# Autodesk Inventor assembly: Сборка1
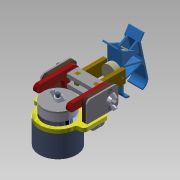
[picture p0: Inventor's stored thumbnail of the model, 180x180]
Saved by Autodesk Inventor 2018 (Build 220112000, 112)
## iProperties
Created: 2020-02-22
Part Number: Сборка1
Material: Типовые
Document SubType Name: Assembly
Designer: Leancher
Mass: 129.322 g
Surface Area: 473.979 cm^2
Volume: 129.322 cm^3
Density: 1 g/cm^3
Author: Leancher
## Documents named in this file (19)
- C:\Users\Leancher\GoogleDrive\My_project\Механика\Фотоштатив\Сборка1.iam
- C:\Users\Leancher\GoogleDrive\My_project\Механика\Фотоштатив\Гор. шарнир.ipt
- C:\Users\Leancher\GoogleDrive\My_project\Механика\Фотоштатив\Верт. держатели.ipt
- C:\Users\Leancher\GoogleDrive\My_project\Механика\Фотоштатив\В.шарн. - втулка.ipt
- C:\Users\Leancher\GoogleDrive\My_project\Механика\Фотоштатив\В. шарн. - держатель соединителя.ipt
- C:\Users\Leancher\GoogleDrive\My_project\Механика\Фотоштатив\В. шарн. - соединитель.ipt
- C:\Users\Leancher\GoogleDrive\My_project\Механика\Фотоштатив\В. шарн. - держатель смартфона.ipt
- C:\Users\Leancher\GoogleDrive\My_project\Механика\Фотоштатив\Чертежи\Гор. шарн. - проставка 1.ipt
- C:\Users\Leancher\GoogleDrive\My_project\Механика\Фотоштатив\Чертежи\Гор. шарн. - прижим.ipt
- C:\Users\Leancher\GoogleDrive\My_project\Механика\Фотоштатив\Чертежи\Верх. часть штатива.ipt
- C:\Users\Leancher\GoogleDrive\My_project\Механика\Фотоштатив\Винт М3х10.ipt
- C:\Users\Leancher\GoogleDrive\My_project\Механика\Фотоштатив\Болт М5х16.ipt
- C:\Users\Leancher\GoogleDrive\My_project\Механика\Фотоштатив\Винт М3х6 пот.ipt
- C:\Users\Leancher\GoogleDrive\My_project\Механика\Фотоштатив\Верт держатели-2 левый.ipt
- C:\Users\Leancher\GoogleDrive\My_project\Механика\Фотоштатив\Верт держатели-2 правый.ipt
- C:\Users\Leancher\GoogleDrive\My_project\Механика\Фотоштатив\Гайка М3.ipt
- C:\Users\Leancher\GoogleDrive\My_project\Механика\Фотоштатив\Гайка-барашек М5.ipt
- C:\Users\Leancher\GoogleDrive\My_project\Механика\Фотоштатив\Прищепка смартфона.ipt
- C:\Users\Leancher\GoogleDrive\My_project\Механика\Фотоштатив\Винт М3х30.ipt
## Components (31 placed, 18 different names)
1. Гор. шарнир:1 — Заподлицо:1, Заподлицо:3
2. Верт. держатели:1 — Вставка:1, Совмещение:27
3. Верт. держатели:2 — Вставка:2, Совмещение:28
4. В.шарн. - втулка:1 — Вставка:2, Совмещение:6, Совмещение:7, Заподлицо:6, Совмещение:21
5. В.шарн. - втулка:2 — Вставка:1, Совмещение:4, Совмещение:5, Совмещение:19, Совмещение:20, Совмещение:22
6. В. шарн. - держатель соединителя:1 — Совмещение:4, Совмещение:5, Совмещение:11
7. В. шарн. - держатель соединителя:2 — Совмещение:6, Совмещение:7, Совмещение:8, Совмещение:9, Совмещение:10
8. В. шарн. - соединитель:1 — Совмещение:8, Совмещение:9, Совмещение:13, Совмещение:14, Совмещение:15, Совмещение:16
9. В. шарн. - соединитель:2 — Совмещение:10, Совмещение:11
10. В. шарн. - держатель смартфона:1 — Совмещение:13, Совмещение:14, Совмещение:32
11. В. шарн. - держатель смартфона:2 — Совмещение:15, Совмещение:16, Совмещение:33
12. Гор. шарн. - проставка 1:1 — Заподлицо:1, Заподлицо:2
13. Гор. шарн. - прижим:1 — Заподлицо:2, Совмещение:31
14. Верх. часть штатива:1 — Заподлицо:3
15. Винт М3х10:1 — Совмещение:25
16. Болт М5х16:1 — Заподлицо:6
17. Болт М5х16:2 — Совмещение:19, Совмещение:20
18. Винт М3х6 пот:1
19. Винт М3х6 пот:2
20. Верт держатели-2 левый:1 — Совмещение:21, Совмещение:23, Заподлицо:7, Совмещение:24, Заподлицо:8, Совмещение:26, Совмещение:30
21. Верт держатели-2 правый:1 — Совмещение:22, Совмещение:25, Совмещение:29
22. Винт М3х6 пот:3 — Совмещение:23, Заподлицо:7
23. Винт М3х6 пот:4 — Совмещение:24, Заподлицо:8
24. Винт М3х10:2 — Совмещение:26
25. Гайка М3:1 — Совмещение:27
26. Гайка М3:2 — Совмещение:28
27. Гайка-барашек М5:1 — Совмещение:31
28. Гайка-барашек М5:2 — Совмещение:29
29. Гайка-барашек М5:3 — Совмещение:30
30. Прищепка смартфона:1 — Совмещение:32
31. Винт М3х30:1 — Совмещение:33
## Relationships (35: Mate 27, Flush 6, Insert 2)
- Вставка:1 [Insert]: Верт. держатели:1 ↔ В.шарн. - втулка:2
- Вставка:2 [Insert]: Верт. держатели:2 ↔ В.шарн. - втулка:1
- Совмещение:4 [Mate]: В.шарн. - втулка:2 ↔ В. шарн. - держатель соединителя:1
- Совмещение:5 [Mate]: В.шарн. - втулка:2 ↔ В. шарн. - держатель соединителя:1
- Совмещение:6 [Mate]: В.шарн. - втулка:1 ↔ В. шарн. - держатель соединителя:2
- Совмещение:7 [Mate]: В.шарн. - втулка:1 ↔ В. шарн. - держатель соединителя:2
- Совмещение:8 [Mate]: В. шарн. - держатель соединителя:2 ↔ В. шарн. - соединитель:1
- Совмещение:9 [Mate]: В. шарн. - держатель соединителя:2 ↔ В. шарн. - соединитель:1
- Совмещение:10 [Mate]: В. шарн. - держатель соединителя:2 ↔ В. шарн. - соединитель:2
- Совмещение:11 [Mate]: В. шарн. - держатель соединителя:1 ↔ В. шарн. - соединитель:2
- Совмещение:13 [Mate]: В. шарн. - соединитель:1 ↔ В. шарн. - держатель смартфона:1
- Совмещение:14 [Mate]: В. шарн. - соединитель:1 ↔ В. шарн. - держатель смартфона:1
- Совмещение:15 [Mate]: В. шарн. - соединитель:1 ↔ В. шарн. - держатель смартфона:2
- Совмещение:16 [Mate]: В. шарн. - соединитель:1 ↔ В. шарн. - держатель смартфона:2
- Заподлицо:1 [Flush]: Гор. шарнир:1 ↔ Гор. шарн. - проставка 1:1
- Заподлицо:2 [Flush]: Гор. шарн. - проставка 1:1 ↔ Гор. шарн. - прижим:1
- Заподлицо:3 [Flush]: Гор. шарнир:1 ↔ Верх. часть штатива:1
- Заподлицо:6 [Flush]: В.шарн. - втулка:1 ↔ Болт М5х16:1
- Совмещение:19 [Mate]: В.шарн. - втулка:2 ↔ Болт М5х16:2
- Совмещение:20 [Mate]: В.шарн. - втулка:2 ↔ Болт М5х16:2
- Совмещение:21 [Mate]: В.шарн. - втулка:1 ↔ Верт держатели-2 левый:1
- Совмещение:22 [Mate]: В.шарн. - втулка:2 ↔ Верт держатели-2 правый:1
- Совмещение:23 [Mate]: Верт держатели-2 левый:1 ↔ Винт М3х6 пот:3
- Заподлицо:7 [Flush]: Верт держатели-2 левый:1 ↔ Винт М3х6 пот:3
- Совмещение:24 [Mate]: Верт держатели-2 левый:1 ↔ Винт М3х6 пот:4
- Заподлицо:8 [Flush]: Верт держатели-2 левый:1 ↔ Винт М3х6 пот:4
- Совмещение:25 [Mate]: Винт М3х10:1 ↔ Верт держатели-2 правый:1
- Совмещение:26 [Mate]: Верт держатели-2 левый:1 ↔ Винт М3х10:2
- Совмещение:27 [Mate]: Верт. держатели:1 ↔ Гайка М3:1
- Совмещение:28 [Mate]: Верт. держатели:2 ↔ Гайка М3:2
- Совмещение:29 [Mate]: Верт держатели-2 правый:1 ↔ Гайка-барашек М5:2
- Совмещение:30 [Mate]: Верт держатели-2 левый:1 ↔ Гайка-барашек М5:3
- Совмещение:31 [Mate]: Гор. шарн. - прижим:1 ↔ Гайка-барашек М5:1
- Совмещение:32 [Mate]: В. шарн. - держатель смартфона:1 ↔ Прищепка смартфона:1
- Совмещение:33 [Mate]: В. шарн. - держатель смартфона:2 ↔ Винт М3х30:1
